# Autodesk Inventor assembly: chess-set-one
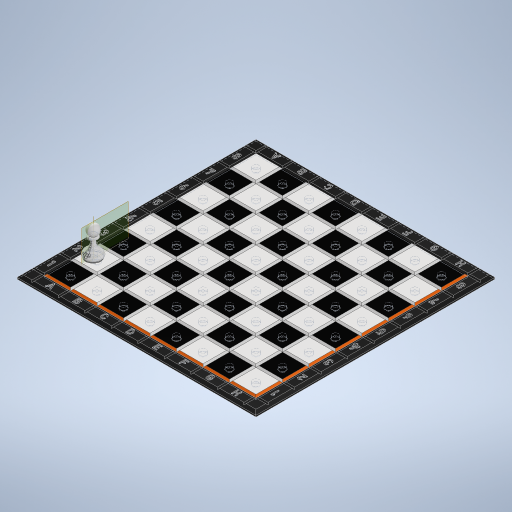
[picture p0: Inventor's stored thumbnail of the model, 512x512]
Saved by Autodesk Inventor 2024.1 (Build 281209000, 209)
## iProperties
Created: 2025-07-31
Part Number: chess-set-one
Document SubType Name: Assembly
Designer: iwheard
Author: iwheard
## Documents named in this file (3)
- C:\Users\iwheard\Documents\0004-CAD\3D-cad-main\chess-set\chess-set-one.iam
- C:\Users\iwheard\Documents\0004-CAD\3D-cad-main\chess-set\board.ipt
- C:\Users\iwheard\Documents\0004-CAD\3D-cad-main\chess-set\pawn-white-v2.ipt
## Components (2 placed, 2 different names)
1. board:1 — Mate:1, Angle:1
2. pawn-white-v2:1 — Mate:1, Angle:1
## Relationships (2: Mate 1, Angle 1)
- Mate:1: board:1 ↔ pawn-white-v2:1
- Angle:1 (0 deg): board:1 ↔ pawn-white-v2:1
